# Autodesk Inventor assembly: 齿轮120
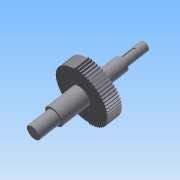
[picture p0: Inventor's stored thumbnail of the model, 180x180]
Saved by Autodesk Inventor 2015 (Build 190159000, 159)
## iProperties
Created: 2017-05-27
Part Number: 齿轮120
Document SubType Name: Assembly
Designer: Administrator
Author: Administrator
## Documents named in this file (3)
- C:\Users\Administrator\Desktop\毕设改\齿轮120.iam
- C:\Users\Administrator\Desktop\毕设改\齿轮120\设计加速器\齿轮1201.iam
- C:\Users\Administrator\Desktop\毕设改\齿轮160配件.ipt
## Components (2 placed, 2 different names)
1. 齿轮120:1 [sub-assembly] — 刚性:1
2. 齿轮160配件:1 — 刚性:1
## Relationships (1: WeldJoint 1)
- 刚性:1 [WeldJoint]: 齿轮120:1 ↔ 齿轮160配件:1
